# Autodesk Inventor assembly: Display
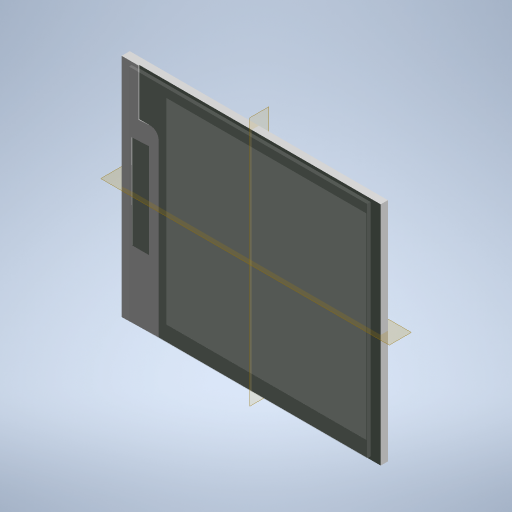
[picture p0: Inventor's stored thumbnail of the model, 512x512]
Saved by Autodesk Inventor 2023 (Build 270158000, 158)
## iProperties
Part Number: Display
Document SubType Name: Assembly
Designer: nigel
Author: nigel
## Documents named in this file (3)
- D:\NIGEL\Documents\GitHub\Watchy-CAD\CAD\Base Model\Display_Touchscreen.iam
- D:\NIGEL\Documents\GitHub\Watchy-CAD\CAD\Base Model\Dsiplay_Touchscreen.ipt
- D:\NIGEL\Documents\GitHub\Watchy-CAD\CAD\Base Model\touch_panel.ipt
## Components (2 placed, 2 different names)
1. Dsiplay_Touchscreen:1 — Mate:1, Mate:2, Flush:1
2. touch_panel:1 — Mate:1, Mate:2, Flush:1
## Relationships (3: Mate 2, Flush 1)
- Mate:1: Dsiplay_Touchscreen:1 ↔ touch_panel:1
- Mate:2: Dsiplay_Touchscreen:1 ↔ touch_panel:1
- Flush:1: Dsiplay_Touchscreen:1 ↔ touch_panel:1
